# Autodesk Inventor assembly: axis_module
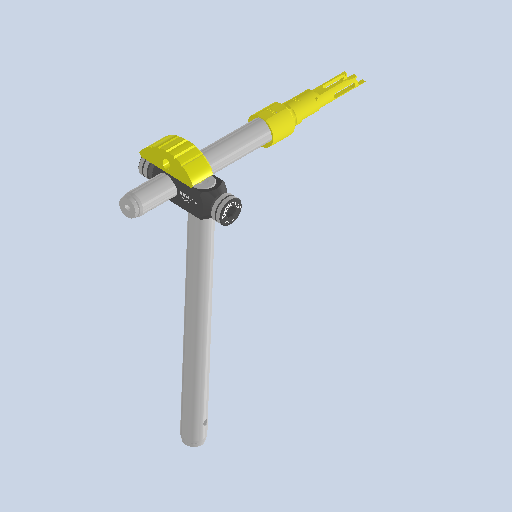
[picture p0: Inventor's stored thumbnail of the model, 512x512]
Saved by Autodesk Inventor 2024 (Build 280153000, 153)
## iProperties
Created: 2021-02-07
Part Number: axis_module
Document SubType Name: Assembly
Designer: dsdan
Author: dsdan
## Documents named in this file (6)
- E:\OneDrive - Imperial College London\DragonVision_DanielKo\Instrumentation\Ephys_rig_2021\axis_module.iam
- E:\OneDrive - Imperial College London\DragonVision_DanielKo\Instrumentation\Ephys_rig_2021\Imported Components\TR100_M-Solidworks.ipt
- E:\OneDrive - Imperial College London\DragonVision_DanielKo\Instrumentation\Ephys_rig_2021\tool_adapter_3.ipt
- E:\OneDrive - Imperial College London\DragonVision_DanielKo\Instrumentation\Ephys_rig_2021\Imported Components\RA90_M-Solidworks.ipt
- E:\OneDrive - Imperial College London\DragonVision_DanielKo\Instrumentation\Ephys_rig_2021\Holder\body_adjustable_parametric_thorlabs.ipt
- E:\OneDrive - Imperial College London\DragonVision_DanielKo\Instrumentation\Ephys_rig_2021\Imported Components\TR150_M-Solidworks\TR150_M-Solidworks.ipt
## Components (5 placed, 5 different names)
1. TR100_M-Solidworks:1 — Mate:5, Mate:6, Mate:42, Mate:52, Mate:53, Mate:54, Mate:55
2. body_adjustable_parametric_thorlabs:1 — Mate:5, Mate:6, Angle:2
3. RA90_M-Solidworks:1 — Mate:48, Flush:50, Flush:51, Mate:52, Angle:1, Mate:54, Angle:2, Mate:56, Flush:52
4. TR150_M-Solidworks:1 — Mate:48, Flush:50, Mate:56, Flush:52
5. tool_adapter_3:1 — Flush:51, Mate:53, Angle:1
## Relationships (14: Mate 9, Flush 3, Angle 2)
- Mate:5: TR100_M-Solidworks:1 ↔ body_adjustable_parametric_thorlabs:1
- Mate:6: TR100_M-Solidworks:1 ↔ body_adjustable_parametric_thorlabs:1
- Mate:42: TR100_M-Solidworks:1
- Mate:48: RA90_M-Solidworks:1 ↔ TR150_M-Solidworks:1
- Flush:50: RA90_M-Solidworks:1 ↔ TR150_M-Solidworks:1
- Flush:51: RA90_M-Solidworks:1 ↔ tool_adapter_3:1
- Mate:52: TR100_M-Solidworks:1 ↔ RA90_M-Solidworks:1
- Mate:53: TR100_M-Solidworks:1 ↔ tool_adapter_3:1
- Angle:1 (180 deg): RA90_M-Solidworks:1 ↔ tool_adapter_3:1
- Mate:54 (-75 mm): TR100_M-Solidworks:1 ↔ RA90_M-Solidworks:1
- Angle:2 (180 deg): body_adjustable_parametric_thorlabs:1 ↔ RA90_M-Solidworks:1
- Mate:55: TR100_M-Solidworks:1
- Mate:56: RA90_M-Solidworks:1 ↔ TR150_M-Solidworks:1
- Flush:52: RA90_M-Solidworks:1 ↔ TR150_M-Solidworks:1
